# Autodesk Inventor assembly: MAIN
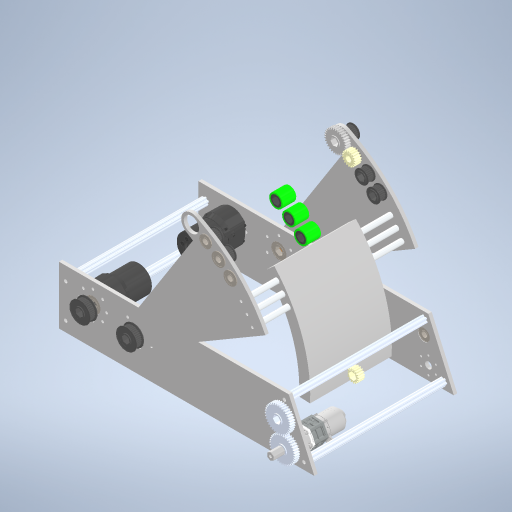
[picture p0: Inventor's stored thumbnail of the model, 512x512]
Saved by Autodesk Inventor 2023 (Build 270158000, 158)
## iProperties
Created: 2023-10-20
Part Number: MAIN
Document SubType Name: Assembly
Designer: jackc
Author: jackc
## Documents named in this file (20)
- C:\Users\jackc\OneDrive\CAD\Parametric Turret\MAIN.iam
- C:\Users\jackc\OneDrive\CAD\Parametric Turret\Flat\Bottom Part.ipt
- C:\Users\jackc\OneDrive\CAD\Parametric Turret\Gears and Pulleys\HoodGearSmooth.ipt
- C:\Users\jackc\OneDrive\CAD\Parametric Turret\Parameters.ipt
- C:\Users\jackc\OneDrive\CAD\Parametric Turret\Motors\NEO Vortex & SPARK Flex (REV-21-1652 & REV-11-2159).ipt
- C:\Users\jackc\OneDrive\CAD\Parametric Turret\0.500 Hex ID x 1.125 OD x 0.313 WD (Flanged Bearing v2) (217-3875).ipt
- C:\Users\jackc\OneDrive\CAD\Parametric Turret\Colson Performa 4 x 1.5, 1_2 Hex bore (217-4052).ipt
- C:\Users\jackc\OneDrive\CAD\Parametric Turret\Gears and Pulleys\UltraPlanetary\REV-41-1600.iam
- C:\Users\jackc\OneDrive\CAD\Parametric Turret\Gears and Pulleys\16t 20dp.ipt
- C:\Users\jackc\OneDrive\CAD\Parametric Turret\Gears and Pulleys\36T Aluminum Spur Gear (20 DP, 1_2 Hex Bore) (217-3214).ipt
- C:\Users\jackc\OneDrive\CAD\Parametric Turret\Gears and Pulleys\36T x 9mm Wide Double Flange Aluminum Pulley (GT2 3mm, 1_2 Hex Bore) (217-5873).ipt
- C:\Users\jackc\OneDrive\CAD\Parametric Turret\Flat\Shooter Side.ipt
- C:\Users\jackc\OneDrive\CAD\Parametric Turret\Gears and Pulleys\10.25mm (3_8 ThunderHex) ID x 0.875 OD x 0.280 WD (Flanged Bearing) (217-5829).ipt
- C:\Users\jackc\OneDrive\CAD\Parametric Turret\Gears and Pulleys\13.75mm (1_2 ThunderHex) ID x 0.625 OD x 0.313 WD (Bronze Flanged Bushing) (217-7348).ipt
- C:\Users\jackc\OneDrive\CAD\Parametric Turret\Gears and Pulleys\am-4541 Sushi Roller 500 Hex Bore.ipt
- C:\Users\jackc\OneDrive\CAD\Parametric Turret\Gears and Pulleys\24T x 9mm Wide Double Flange Aluminum Pulley (GT2 3mm, 1_2 Hex Bore) (217-5875).ipt
- C:\Users\jackc\OneDrive\CAD\Parametric Turret\Gears and Pulleys\18T Aluminum Spur Gear (20 DP, 3_8 Hex Bore) (217-3208).ipt
- C:\Users\jackc\OneDrive\CAD\Parametric Turret\Gears and Pulleys\30T Aluminum Spur Gear (20 DP, 1_2 Hex Bore) (217-2705).ipt
- C:\Users\jackc\OneDrive\CAD\Parametric Turret\Stock\MainChurro.ipt
- C:\Users\jackc\OneDrive\CAD\Parametric Turret\Stock\Hood Support 3_8 Tube.ipt
## Components (47 placed, 18 different names)
1. Bottom Part:1 — Mate:1, Flush:1, Flush:2, Mate:8, Mate:11, Mate:86, Mate:99, Mate:100
2. Bottom Part:2 — Mate:1, Mate:2, Mate:3, Flush:1, Flush:2, Mate:5, Mate:6, Mate:9, Mate:10, Mate:13, Mate:14, Mate:15, Mate:24, Mate:27, Mate:87, Mate:88, Mate:89, Mate:90, Mate:91, Mate:98, Mate:102, Mate:103
3. HoodGearSmooth:1 — Mate:2, Mate:3, Mate:30, Mate:31, Mate:34, Flush:11, Flush:12
4. NEO Vortex & SPARK Flex (REV-21-1652 & REV-11-2159):1 — Mate:81, Mate:83, Mate:84, Mate:86
5. NEO Vortex & SPARK Flex (REV-21-1652 & REV-11-2159):2 — Mate:5, Mate:6, Mate:81
6. 0.500 Hex ID x 1.125 OD x 0.313 WD (Flanged Bearing v2) (217-3875):1 — Mate:8, Mate:11, Mate:12, Mate:32, Mate:40
7. 0.500 Hex ID x 1.125 OD x 0.313 WD (Flanged Bearing v2) (217-3875):2 — Mate:9, Mate:10, Mate:29, Mate:33, Mate:39
8. Colson Performa 4 x 1.5, 1_2 Hex bore (217-4052):1 — Mate:12, Mate:13
9. REV-41-1600:1 [sub-assembly] — Mate:14, Mate:15, Mate:21
10. 16t 20dp:1 — Flush:11, Mate:102
11. 36T Aluminum Spur Gear (20 DP, 1_2 Hex Bore) (217-3214):1 — Mate:21, Flush:3
12. 36T Aluminum Spur Gear (20 DP, 1_2 Hex Bore) (217-3214):2 — Flush:3, Mate:101
13. 0.500 Hex ID x 1.125 OD x 0.313 WD (Flanged Bearing v2) (217-3875):5 — Mate:24, Mate:27, Mate:28
14. 0.500 Hex ID x 1.125 OD x 0.313 WD (Flanged Bearing v2) (217-3875):6 — Mate:83, Mate:84
15. 36T x 9mm Wide Double Flange Aluminum Pulley (GT2 3mm, 1_2 Hex Bore) (217-5873):1 — Mate:28, Flush:4
16. 36T x 9mm Wide Double Flange Aluminum Pulley (GT2 3mm, 1_2 Hex Bore) (217-5873):2 — Mate:29, Flush:4, Mate:60
17. Shooter Side:1 — Mate:31, Mate:32, Mate:35, Mate:36, Mate:41, Mate:42, Mate:43, Mate:49, Mate:50, Mate:51, Mate:53, Mate:59, Mate:92, Mate:94, Mate:95, Mate:96, Mate:97
18. Shooter Side:2 — Mate:30, Mate:33, Mate:34, Mate:37, Mate:38, Mate:44, Mate:45, Mate:46, Mate:47, Mate:48, Mate:93
19. 10.25mm (3_8 ThunderHex) ID x 0.875 OD x 0.280 WD (Flanged Bearing) (217-5829):1 — Mate:41, Mate:49, Mate:56, Mate:78
20. 13.75mm (1_2 ThunderHex) ID x 0.625 OD x 0.313 WD (Bronze Flanged Bushing) (217-7348):1 — Mate:35, Mate:36, Mate:40, Mate:80
21. am-4541 Sushi Roller 500 Hex Bore:1 — Mate:56, Flush:6
22. 13.75mm (1_2 ThunderHex) ID x 0.625 OD x 0.313 WD (Bronze Flanged Bushing) (217-7348):2 — Mate:37, Mate:38, Mate:39, Mate:60
23. 10.25mm (3_8 ThunderHex) ID x 0.875 OD x 0.280 WD (Flanged Bearing) (217-5829):2 — Mate:42, Mate:50, Mate:57, Mate:65
24. 10.25mm (3_8 ThunderHex) ID x 0.875 OD x 0.280 WD (Flanged Bearing) (217-5829):3 — Mate:43, Mate:51, Mate:58, Mate:70
25. 10.25mm (3_8 ThunderHex) ID x 0.875 OD x 0.280 WD (Flanged Bearing) (217-5829):4 — Mate:44, Flush:5, Mate:74, Mate:85
26. 10.25mm (3_8 ThunderHex) ID x 0.875 OD x 0.280 WD (Flanged Bearing) (217-5829):5 — Mate:45, Flush:5, Mate:47, Mate:75
27. 10.25mm (3_8 ThunderHex) ID x 0.875 OD x 0.280 WD (Flanged Bearing) (217-5829):6 — Mate:46, Mate:48
28. 0.500 Hex ID x 1.125 OD x 0.313 WD (Flanged Bearing v2) (217-3875):7 — Mate:53, Mate:59, Mate:67, Mate:77, Mate:79
29. am-4541 Sushi Roller 500 Hex Bore:2 — Mate:57, Flush:6, Flush:7, Flush:12
30. am-4541 Sushi Roller 500 Hex Bore:3 — Mate:58, Flush:7
31. 24T x 9mm Wide Double Flange Aluminum Pulley (GT2 3mm, 1_2 Hex Bore) (217-5875):1 — Flush:9, Mate:80
32. 24T x 9mm Wide Double Flange Aluminum Pulley (GT2 3mm, 1_2 Hex Bore) (217-5875):2 — Flush:9, Mate:73, Mate:79
33. 24T x 9mm Wide Double Flange Aluminum Pulley (GT2 3mm, 1_2 Hex Bore) (217-5875):3 — Mate:74, Flush:10, Mate:85
34. 24T x 9mm Wide Double Flange Aluminum Pulley (GT2 3mm, 1_2 Hex Bore) (217-5875):4 — Mate:75, Flush:10
35. 24T x 9mm Wide Double Flange Aluminum Pulley (GT2 3mm, 1_2 Hex Bore) (217-5875):5 — Mate:65, Flush:14
36. 24T x 9mm Wide Double Flange Aluminum Pulley (GT2 3mm, 1_2 Hex Bore) (217-5875):6 — Mate:70, Flush:14
37. 18T Aluminum Spur Gear (20 DP, 3_8 Hex Bore) (217-3208):1 — Flush:13, Mate:78
38. 30T Aluminum Spur Gear (20 DP, 1_2 Hex Bore) (217-2705):1 — Mate:67, Mate:73, Mate:77, Flush:13
39. MainChurro:1 — Mate:88, Flush:17
40. MainChurro:2 — Mate:87, Flush:16, Flush:17, Mate:91
41. MainChurro:3 — Mate:89, Flush:15, Flush:16
42. MainChurro:4 — Mate:90, Flush:15
43. Hood Support 3_8 Tube:1 — Mate:92, Mate:93
44. Hood Support 3_8 Tube:2 — Mate:94, Mate:96
45. Hood Support 3_8 Tube:3 — Mate:95, Mate:97
46. 10.25mm (3_8 ThunderHex) ID x 0.875 OD x 0.280 WD (Flanged Bearing) (217-5829):7 — Mate:98, Mate:101, Mate:103
47. 10.25mm (3_8 ThunderHex) ID x 0.875 OD x 0.280 WD (Flanged Bearing) (217-5829):8 — Mate:99, Mate:100
## Relationships (94: Mate 78, Flush 16)
- Mate:1 (254 mm): Bottom Part:1 ↔ Bottom Part:2
- Mate:2: Bottom Part:2 ↔ HoodGearSmooth:1
- Mate:3 (50.8 mm): Bottom Part:2 ↔ HoodGearSmooth:1
- Flush:1: Bottom Part:1 ↔ Bottom Part:2
- Flush:2: Bottom Part:1 ↔ Bottom Part:2
- Mate:5: Bottom Part:2 ↔ NEO Vortex & SPARK Flex (REV-21-1652 & REV-11-2159):2
- Mate:6: Bottom Part:2 ↔ NEO Vortex & SPARK Flex (REV-21-1652 & REV-11-2159):2
- Mate:8: Bottom Part:1 ↔ 0.500 Hex ID x 1.125 OD x 0.313 WD (Flanged Bearing v2) (217-3875):1
- Mate:9: Bottom Part:2 ↔ 0.500 Hex ID x 1.125 OD x 0.313 WD (Flanged Bearing v2) (217-3875):2
- Mate:10: Bottom Part:2 ↔ 0.500 Hex ID x 1.125 OD x 0.313 WD (Flanged Bearing v2) (217-3875):2
- Mate:11: Bottom Part:1 ↔ 0.500 Hex ID x 1.125 OD x 0.313 WD (Flanged Bearing v2) (217-3875):1
- Mate:12: 0.500 Hex ID x 1.125 OD x 0.313 WD (Flanged Bearing v2) (217-3875):1 ↔ Colson Performa 4 x 1.5, 1_2 Hex bore (217-4052):1
- Mate:13 (105.5545 mm): Bottom Part:2 ↔ Colson Performa 4 x 1.5, 1_2 Hex bore (217-4052):1
- Mate:14: Bottom Part:2 ↔ REV-41-1600:1
- Mate:15 (10.16 mm): Bottom Part:2 ↔ REV-41-1600:1
- Mate:21: REV-41-1600:1 ↔ 36T Aluminum Spur Gear (20 DP, 1_2 Hex Bore) (217-3214):1
- Flush:3: 36T Aluminum Spur Gear (20 DP, 1_2 Hex Bore) (217-3214):1 ↔ 36T Aluminum Spur Gear (20 DP, 1_2 Hex Bore) (217-3214):2
- Mate:24: Bottom Part:2 ↔ 0.500 Hex ID x 1.125 OD x 0.313 WD (Flanged Bearing v2) (217-3875):5
- Mate:27: Bottom Part:2 ↔ 0.500 Hex ID x 1.125 OD x 0.313 WD (Flanged Bearing v2) (217-3875):5
- Mate:28: 0.500 Hex ID x 1.125 OD x 0.313 WD (Flanged Bearing v2) (217-3875):5 ↔ 36T x 9mm Wide Double Flange Aluminum Pulley (GT2 3mm, 1_2 Hex Bore) (217-5873):1
- Mate:29: 0.500 Hex ID x 1.125 OD x 0.313 WD (Flanged Bearing v2) (217-3875):2 ↔ 36T x 9mm Wide Double Flange Aluminum Pulley (GT2 3mm, 1_2 Hex Bore) (217-5873):2
- Flush:4: 36T x 9mm Wide Double Flange Aluminum Pulley (GT2 3mm, 1_2 Hex Bore) (217-5873):1 ↔ 36T x 9mm Wide Double Flange Aluminum Pulley (GT2 3mm, 1_2 Hex Bore) (217-5873):2
- Mate:30: HoodGearSmooth:1 ↔ Shooter Side:2
- Mate:31: HoodGearSmooth:1 ↔ Shooter Side:1
- Mate:32: 0.500 Hex ID x 1.125 OD x 0.313 WD (Flanged Bearing v2) (217-3875):1 ↔ Shooter Side:1
- Mate:33: 0.500 Hex ID x 1.125 OD x 0.313 WD (Flanged Bearing v2) (217-3875):2 ↔ Shooter Side:2
- Mate:34: HoodGearSmooth:1 ↔ Shooter Side:2
- Mate:35: Shooter Side:1 ↔ 13.75mm (1_2 ThunderHex) ID x 0.625 OD x 0.313 WD (Bronze Flanged Bushing) (217-7348):1
- Mate:36: Shooter Side:1 ↔ 13.75mm (1_2 ThunderHex) ID x 0.625 OD x 0.313 WD (Bronze Flanged Bushing) (217-7348):1
- Mate:37: Shooter Side:2 ↔ 13.75mm (1_2 ThunderHex) ID x 0.625 OD x 0.313 WD (Bronze Flanged Bushing) (217-7348):2
- Mate:38: Shooter Side:2 ↔ 13.75mm (1_2 ThunderHex) ID x 0.625 OD x 0.313 WD (Bronze Flanged Bushing) (217-7348):2
- Mate:39: 0.500 Hex ID x 1.125 OD x 0.313 WD (Flanged Bearing v2) (217-3875):2 ↔ 13.75mm (1_2 ThunderHex) ID x 0.625 OD x 0.313 WD (Bronze Flanged Bushing) (217-7348):2
- Mate:40: 0.500 Hex ID x 1.125 OD x 0.313 WD (Flanged Bearing v2) (217-3875):1 ↔ 13.75mm (1_2 ThunderHex) ID x 0.625 OD x 0.313 WD (Bronze Flanged Bushing) (217-7348):1
- Mate:41: Shooter Side:1 ↔ 10.25mm (3_8 ThunderHex) ID x 0.875 OD x 0.280 WD (Flanged Bearing) (217-5829):1
- Mate:42: Shooter Side:1 ↔ 10.25mm (3_8 ThunderHex) ID x 0.875 OD x 0.280 WD (Flanged Bearing) (217-5829):2
- Mate:43: Shooter Side:1 ↔ 10.25mm (3_8 ThunderHex) ID x 0.875 OD x 0.280 WD (Flanged Bearing) (217-5829):3
- Mate:44: Shooter Side:2 ↔ 10.25mm (3_8 ThunderHex) ID x 0.875 OD x 0.280 WD (Flanged Bearing) (217-5829):4
- Mate:45: Shooter Side:2 ↔ 10.25mm (3_8 ThunderHex) ID x 0.875 OD x 0.280 WD (Flanged Bearing) (217-5829):5
- Mate:46: Shooter Side:2 ↔ 10.25mm (3_8 ThunderHex) ID x 0.875 OD x 0.280 WD (Flanged Bearing) (217-5829):6
- Flush:5: 10.25mm (3_8 ThunderHex) ID x 0.875 OD x 0.280 WD (Flanged Bearing) (217-5829):4 ↔ 10.25mm (3_8 ThunderHex) ID x 0.875 OD x 0.280 WD (Flanged Bearing) (217-5829):5
- Mate:47: Shooter Side:2 ↔ 10.25mm (3_8 ThunderHex) ID x 0.875 OD x 0.280 WD (Flanged Bearing) (217-5829):5
- Mate:48: Shooter Side:2 ↔ 10.25mm (3_8 ThunderHex) ID x 0.875 OD x 0.280 WD (Flanged Bearing) (217-5829):6
- Mate:49: Shooter Side:1 ↔ 10.25mm (3_8 ThunderHex) ID x 0.875 OD x 0.280 WD (Flanged Bearing) (217-5829):1
- Mate:50: Shooter Side:1 ↔ 10.25mm (3_8 ThunderHex) ID x 0.875 OD x 0.280 WD (Flanged Bearing) (217-5829):2
- Mate:51: Shooter Side:1 ↔ 10.25mm (3_8 ThunderHex) ID x 0.875 OD x 0.280 WD (Flanged Bearing) (217-5829):3
- Mate:53: Shooter Side:1 ↔ 0.500 Hex ID x 1.125 OD x 0.313 WD (Flanged Bearing v2) (217-3875):7
- Mate:56: 10.25mm (3_8 ThunderHex) ID x 0.875 OD x 0.280 WD (Flanged Bearing) (217-5829):1 ↔ am-4541 Sushi Roller 500 Hex Bore:1
- Mate:57: 10.25mm (3_8 ThunderHex) ID x 0.875 OD x 0.280 WD (Flanged Bearing) (217-5829):2 ↔ am-4541 Sushi Roller 500 Hex Bore:2
- Mate:58: 10.25mm (3_8 ThunderHex) ID x 0.875 OD x 0.280 WD (Flanged Bearing) (217-5829):3 ↔ am-4541 Sushi Roller 500 Hex Bore:3
- Flush:6: am-4541 Sushi Roller 500 Hex Bore:1 ↔ am-4541 Sushi Roller 500 Hex Bore:2
- Flush:7: am-4541 Sushi Roller 500 Hex Bore:2 ↔ am-4541 Sushi Roller 500 Hex Bore:3
- Mate:59: Shooter Side:1 ↔ 0.500 Hex ID x 1.125 OD x 0.313 WD (Flanged Bearing v2) (217-3875):7
- Mate:60: 36T x 9mm Wide Double Flange Aluminum Pulley (GT2 3mm, 1_2 Hex Bore) (217-5873):2 ↔ 13.75mm (1_2 ThunderHex) ID x 0.625 OD x 0.313 WD (Bronze Flanged Bushing) (217-7348):2
- Mate:65: 10.25mm (3_8 ThunderHex) ID x 0.875 OD x 0.280 WD (Flanged Bearing) (217-5829):2 ↔ 24T x 9mm Wide Double Flange Aluminum Pulley (GT2 3mm, 1_2 Hex Bore) (217-5875):5
- Mate:67: 0.500 Hex ID x 1.125 OD x 0.313 WD (Flanged Bearing v2) (217-3875):7 ↔ 30T Aluminum Spur Gear (20 DP, 1_2 Hex Bore) (217-2705):1
- Mate:70: 10.25mm (3_8 ThunderHex) ID x 0.875 OD x 0.280 WD (Flanged Bearing) (217-5829):3 ↔ 24T x 9mm Wide Double Flange Aluminum Pulley (GT2 3mm, 1_2 Hex Bore) (217-5875):6
- Flush:9: 24T x 9mm Wide Double Flange Aluminum Pulley (GT2 3mm, 1_2 Hex Bore) (217-5875):1 ↔ 24T x 9mm Wide Double Flange Aluminum Pulley (GT2 3mm, 1_2 Hex Bore) (217-5875):2
- Mate:73: 24T x 9mm Wide Double Flange Aluminum Pulley (GT2 3mm, 1_2 Hex Bore) (217-5875):2 ↔ 30T Aluminum Spur Gear (20 DP, 1_2 Hex Bore) (217-2705):1
- Mate:74: 10.25mm (3_8 ThunderHex) ID x 0.875 OD x 0.280 WD (Flanged Bearing) (217-5829):4 ↔ 24T x 9mm Wide Double Flange Aluminum Pulley (GT2 3mm, 1_2 Hex Bore) (217-5875):3
- Mate:75: 10.25mm (3_8 ThunderHex) ID x 0.875 OD x 0.280 WD (Flanged Bearing) (217-5829):5 ↔ 24T x 9mm Wide Double Flange Aluminum Pulley (GT2 3mm, 1_2 Hex Bore) (217-5875):4
- Flush:10: 24T x 9mm Wide Double Flange Aluminum Pulley (GT2 3mm, 1_2 Hex Bore) (217-5875):3 ↔ 24T x 9mm Wide Double Flange Aluminum Pulley (GT2 3mm, 1_2 Hex Bore) (217-5875):4
- Flush:11 (69.8754 mm): HoodGearSmooth:1 ↔ 16t 20dp:1
- Flush:12 (63.5 mm): HoodGearSmooth:1 ↔ am-4541 Sushi Roller 500 Hex Bore:2
- Mate:77: 0.500 Hex ID x 1.125 OD x 0.313 WD (Flanged Bearing v2) (217-3875):7 ↔ 30T Aluminum Spur Gear (20 DP, 1_2 Hex Bore) (217-2705):1
- Flush:13: 18T Aluminum Spur Gear (20 DP, 3_8 Hex Bore) (217-3208):1 ↔ 30T Aluminum Spur Gear (20 DP, 1_2 Hex Bore) (217-2705):1
- Mate:78: 10.25mm (3_8 ThunderHex) ID x 0.875 OD x 0.280 WD (Flanged Bearing) (217-5829):1 ↔ 18T Aluminum Spur Gear (20 DP, 3_8 Hex Bore) (217-3208):1
- Mate:79: 0.500 Hex ID x 1.125 OD x 0.313 WD (Flanged Bearing v2) (217-3875):7 ↔ 24T x 9mm Wide Double Flange Aluminum Pulley (GT2 3mm, 1_2 Hex Bore) (217-5875):2
- Mate:80: 13.75mm (1_2 ThunderHex) ID x 0.625 OD x 0.313 WD (Bronze Flanged Bushing) (217-7348):1 ↔ 24T x 9mm Wide Double Flange Aluminum Pulley (GT2 3mm, 1_2 Hex Bore) (217-5875):1
- Mate:81: NEO Vortex & SPARK Flex (REV-21-1652 & REV-11-2159):1 ↔ NEO Vortex & SPARK Flex (REV-21-1652 & REV-11-2159):2
- Mate:83: NEO Vortex & SPARK Flex (REV-21-1652 & REV-11-2159):1 ↔ 0.500 Hex ID x 1.125 OD x 0.313 WD (Flanged Bearing v2) (217-3875):6
- Mate:84: NEO Vortex & SPARK Flex (REV-21-1652 & REV-11-2159):1 ↔ 0.500 Hex ID x 1.125 OD x 0.313 WD (Flanged Bearing v2) (217-3875):6
- Flush:14: 24T x 9mm Wide Double Flange Aluminum Pulley (GT2 3mm, 1_2 Hex Bore) (217-5875):5 ↔ 24T x 9mm Wide Double Flange Aluminum Pulley (GT2 3mm, 1_2 Hex Bore) (217-5875):6
- Mate:85: 10.25mm (3_8 ThunderHex) ID x 0.875 OD x 0.280 WD (Flanged Bearing) (217-5829):4 ↔ 24T x 9mm Wide Double Flange Aluminum Pulley (GT2 3mm, 1_2 Hex Bore) (217-5875):3
- Mate:86: Bottom Part:1 ↔ NEO Vortex & SPARK Flex (REV-21-1652 & REV-11-2159):1
- Mate:87: Bottom Part:2 ↔ MainChurro:2
- Mate:88: Bottom Part:2 ↔ MainChurro:1
- Mate:89: Bottom Part:2 ↔ MainChurro:3
- Mate:90: Bottom Part:2 ↔ MainChurro:4
- Flush:15: MainChurro:3 ↔ MainChurro:4
- Flush:16: MainChurro:2 ↔ MainChurro:3
- Flush:17: MainChurro:1 ↔ MainChurro:2
- Mate:91: Bottom Part:2 ↔ MainChurro:2
- Mate:92: Shooter Side:1 ↔ Hood Support 3_8 Tube:1
- Mate:93: Shooter Side:2 ↔ Hood Support 3_8 Tube:1
- Mate:94: Shooter Side:1 ↔ Hood Support 3_8 Tube:2
- Mate:95: Shooter Side:1 ↔ Hood Support 3_8 Tube:3
- Mate:96: Shooter Side:1 ↔ Hood Support 3_8 Tube:2
- Mate:97: Shooter Side:1 ↔ Hood Support 3_8 Tube:3
- Mate:98: Bottom Part:2 ↔ 10.25mm (3_8 ThunderHex) ID x 0.875 OD x 0.280 WD (Flanged Bearing) (217-5829):7
- Mate:99: Bottom Part:1 ↔ 10.25mm (3_8 ThunderHex) ID x 0.875 OD x 0.280 WD (Flanged Bearing) (217-5829):8
- Mate:100: Bottom Part:1 ↔ 10.25mm (3_8 ThunderHex) ID x 0.875 OD x 0.280 WD (Flanged Bearing) (217-5829):8
- Mate:101: 36T Aluminum Spur Gear (20 DP, 1_2 Hex Bore) (217-3214):2 ↔ 10.25mm (3_8 ThunderHex) ID x 0.875 OD x 0.280 WD (Flanged Bearing) (217-5829):7
- Mate:102: Bottom Part:2 ↔ 16t 20dp:1
- Mate:103: Bottom Part:2 ↔ 10.25mm (3_8 ThunderHex) ID x 0.875 OD x 0.280 WD (Flanged Bearing) (217-5829):7
## Named parameters: BallSize1 = 304.8 mm, WheelSize = 101.6 mm, BallSize = 203.2 mm, Compression = 12.7 mm, TeethNumber = 410
